# Autodesk Inventor assembly: casingForHack
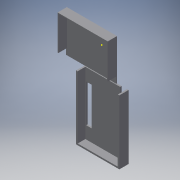
[picture p0: Inventor's stored thumbnail of the model, 180x180]
Saved by Autodesk Inventor 2017 (Build 210142000, 142)
## iProperties
Created: 2018-02-18
Part Number: casingForHack
Document SubType Name: Assembly
Designer: Jacob
Author: Jacob
## Documents named in this file (3)
- C:\Users\Jacob\Desktop\casingForHack.iam
- C:\Users\Jacob\Desktop\Part4.ipt
- C:\Users\Jacob\Documents\Breadboard case.ipt
## Components (2 placed, 2 different names)
1. Part4:1 — Mate:1, Flush:1, Flush:2
2. Breadboard case:1 — Mate:1, Flush:1, Flush:2
## Relationships (3: Flush 2, Mate 1)
- Mate:1: Part4:1 ↔ Breadboard case:1
- Flush:1: Part4:1 ↔ Breadboard case:1
- Flush:2 (15 mm): Part4:1 ↔ Breadboard case:1
